# Autodesk Inventor assembly: SensorLamp_new
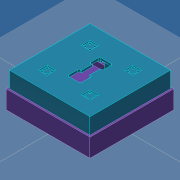
[picture p0: Inventor's stored thumbnail of the model, 180x180]
Saved by Autodesk Inventor 2016 SP2 (Build 200236200, 236)
## iProperties
Created: 2017-11-26
Part Number: SensorLamp_new
Material: Generisch
Document SubType Name: Assembly
Designer: User
Author: User
## Documents named in this file (4)
- C:\Users\User\Documents\Inventor\SensorLamp\SensorLamp_new.iam
- C:\Users\User\Documents\Inventor\SensorLamp\Sensorlamp_Base_new.ipt
- C:\Users\User\Documents\Inventor\SensorLamp\PCB_70x30.ipt
- C:\Users\User\Documents\Inventor\SensorLamp\Sensorlamp_Cover_new.ipt
## Components (3 placed, 3 different names)
1. Sensorlamp_Base_new:1 — Passend:1, Passend:3, Passend:4, Fluchtend:1, Fluchtend:2, Passend:5
2. PCB_70x30:1 — Passend:1, Passend:3, Passend:4
3. Sensorlamp_Cover_new:1 — Fluchtend:1, Fluchtend:2, Passend:5
## Relationships (6: Mate 4, Flush 2)
- Passend:1 [Mate]: Sensorlamp_Base_new:1 ↔ PCB_70x30:1
- Passend:3 [Mate]: Sensorlamp_Base_new:1 ↔ PCB_70x30:1
- Passend:4 [Mate]: Sensorlamp_Base_new:1 ↔ PCB_70x30:1
- Fluchtend:1 [Flush]: Sensorlamp_Base_new:1 ↔ Sensorlamp_Cover_new:1
- Fluchtend:2 [Flush]: Sensorlamp_Base_new:1 ↔ Sensorlamp_Cover_new:1
- Passend:5 [Mate]: Sensorlamp_Base_new:1 ↔ Sensorlamp_Cover_new:1
